# Autodesk Inventor assembly: Cooling Mechanism
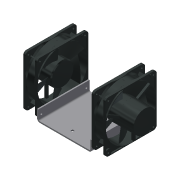
[picture p0: Inventor's stored thumbnail of the model, 180x180]
Saved by Autodesk Inventor 2014 SP1 (Build 180222100, 222)
## iProperties
Created: 2014-11-20
Part Number: Cooling Mechanism
Document SubType Name: Assembly
Designer: AlecShufelt
Author: AlecShufelt
## Documents named in this file (3)
- C:\Users\AlecShufelt\Documents\Drafting\CEMS Research\Prototype 2.0\Cooling Mechanism.iam
- C:\Users\AlecShufelt\Documents\Drafting\CEMS Research\Prototype 2.0\Imported Components\AC4300H_ebm-papst\AC4300H_ebm-papst.iam
- C:\Users\AlecShufelt\Documents\Drafting\CEMS Research\Prototype 2.0\Part156.ipt
## Components (3 placed, 2 different names)
1. Part156:1 — Insert:1
2. AC4300H_ebm-papst:3 [sub-assembly]
3. AC4300H_ebm-papst:4 [sub-assembly] — Insert:1
## Relationships (1: Insert 1)
- Insert:1: Part156:1 ↔ AC4300H_ebm-papst:4
